# Autodesk Inventor assembly: Head
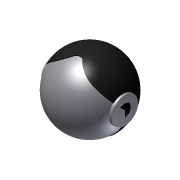
[picture p0: Inventor's stored thumbnail of the model, 180x180]
Saved by Autodesk Inventor 2011 (Build 150239000, 239)
## iProperties
Created: 2011-04-09
Part Number: Head
Document SubType Name: Assembly
Designer: Milton
Author: Milton
## Documents named in this file (3)
- C:\Users\Milton\Documents\Futbots\IC - Humanóide\Desenhos\Head.iam
- C:\Users\Milton\Documents\Futbots\IC - Humanóide\Desenhos\Head.ipt
- C:\Users\Milton\Documents\Futbots\IC - Humanóide\Desenhos\Visor.ipt
## Components (2 placed, 2 different names)
1. Head:1 — Mate:1
2. Visor:1 — Mate:1
## Relationships (1: Mate 1)
- Mate:1: Head:1 ↔ Visor:1
